# Autodesk Inventor assembly: 000.100 - Манипулятор
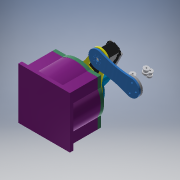
[picture p0: Inventor's stored thumbnail of the model, 180x180]
Saved by Autodesk Inventor 2019 (Build 230136000, 136)
## iProperties
Created: 2020-03-17
Part Number: 000.100 - Манипулятор
Material: Типовые
Document SubType Name: Assembly
Designer: Петров Иван
Author: Петров Иван
## Documents named in this file (4)
- E:\IVAN\Ivan_desktop\GitHub\Manipulation_IRS\hardware\SCARA\000.100 - Манипулятор.iam
- E:\IVAN\Ivan_desktop\GitHub\Manipulation_IRS\hardware\SCARA\000.200 - Основание.iam
- E:\IVAN\Ivan_desktop\GitHub\Manipulation_IRS\hardware\SCARA\000.300 - Рычаг 1.iam
- E:\IVAN\Ivan_desktop\GitHub\Manipulation_IRS\hardware\SCARA\000.400 - Рычаг 2.iam
## Components (3 placed, 3 different names)
1. 000.200 - Основание:1 [sub-assembly] — Совмещение:1, Совмещение:2, Совмещение:3
2. 000.300 - Рычаг 1:1 [sub-assembly] — Совмещение:1, Совмещение:2, Совмещение:3, Совмещение:4, Совмещение:5, Совмещение:6
3. 000.400 - Рычаг 2:1 [sub-assembly] — Совмещение:4, Совмещение:5, Совмещение:6
## Relationships (6: Mate 6)
- Совмещение:1 [Mate]: 000.200 - Основание:1 ↔ 000.300 - Рычаг 1:1
- Совмещение:2 [Mate]: 000.200 - Основание:1 ↔ 000.300 - Рычаг 1:1
- Совмещение:3 [Mate]: 000.200 - Основание:1 ↔ 000.300 - Рычаг 1:1
- Совмещение:4 [Mate]: 000.300 - Рычаг 1:1 ↔ 000.400 - Рычаг 2:1
- Совмещение:5 [Mate]: 000.300 - Рычаг 1:1 ↔ 000.400 - Рычаг 2:1
- Совмещение:6 [Mate]: 000.300 - Рычаг 1:1 ↔ 000.400 - Рычаг 2:1
